# Autodesk Inventor assembly: TankFlipperAssembledDriveShaft
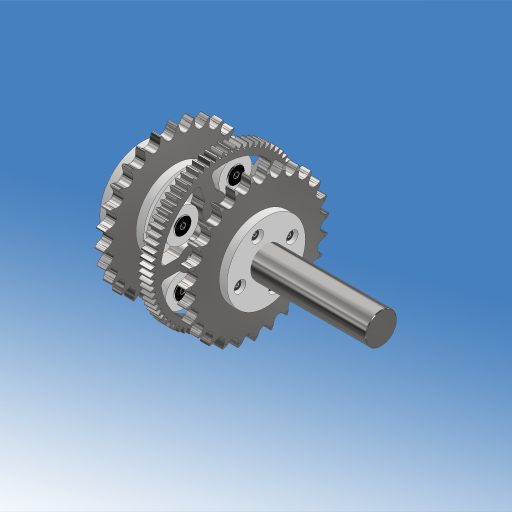
[picture p0: Inventor's stored thumbnail of the model, 512x512]
Saved by Autodesk Inventor 2024 (Build 280153000, 153)
## iProperties
Created: 2024-02-13
Part Number: TankFlipperAssembledDriveShaft
Document SubType Name: Assembly
Designer: seene
Author: seene
## Documents named in this file (12)
- C:\Users\seene\OneDrive\SBRT\Robocup Rescue\Drive\v1\TANK flipper\TankFlipperAssembledDriveShaft.iam
- C:\Users\seene\OneDrive\SBRT\Robocup Rescue\Drive\v1\TANK flipper\Drive Shaft.ipt
- C:\Users\seene\OneDrive\SBRT\Robocup Rescue\Drive\v1\TANK flipper\98585A121_Heavy Duty External Retaining Ring v2.ipt
- C:\Users\seene\OneDrive\SBRT\Robocup Rescue\Drive\v1\TANK flipper\2868T199_High-Load Oil-Embedded 863 Sleeve Bearing (1) v2(Mirror).ipt
- C:\Users\seene\OneDrive\SBRT\Robocup Rescue\Drive\v1\TANK flipper\27t track drive sprocket v25.iam
- C:\Users\seene\OneDrive\SBRT\Robocup Rescue\Drive\v1\TANK flipper\Spur Gear (74 teeth).ipt
- C:\Users\seene\OneDrive\SBRT\Robocup Rescue\Drive\v1\TANK flipper\panel_flange.ipt
- C:\Users\seene\Downloads\SBRT\SBRT\Flipper_assy\spacer_flange.ipt
- C:\Users\seene\OneDrive\SBRT\Robocup Rescue\Drive\v1\TANK flipper\transfer_pin.ipt
- C:\Users\seene\OneDrive\SBRT\Robocup Rescue\Drive\v1\TANK flipper\.25-20_FHCS_91263A553.ipt
- C:\Users\seene\OneDrive\SBRT\Robocup Rescue\Drive\v1\TANK flipper\bushing_2868T199.ipt
- C:\Users\seene\OneDrive\SBRT\Robocup Rescue\Drive\v1\TANK flipper\94328A911_Black Oxide Alloy Steel Low-Profile Shoulder Screw v2.ipt
## Components (29 placed, 11 different names)
1. Drive Shaft:1 — Rigid:1, Rigid:2, Rigid:3, Rigid:4, Rigid:5, Rigid:17
2. 98585A121_Heavy Duty External Retaining Ring v2:1 — Rigid:1
3. 2868T199_High-Load Oil-Embedded 863 Sleeve Bearing (1) v2(Mirror):1 — Rigid:2, Rigid:18
4. 27t track drive sprocket v25:1 [sub-assembly] — Rigid:4
5. 98585A121_Heavy Duty External Retaining Ring v2:2 — Rigid:3
6. 98585A121_Heavy Duty External Retaining Ring v2:3 — Rigid:5
7. Spur Gear (74 teeth):1 — Mate:1, Mate:2, Rigid:16
8. panel_flange:1 — Rigid:18
9. panel_flange:2 — Mate:3, Mate:4, Mate:5, Rigid:25
10. spacer_flange:1 — Rigid:6, Rigid:7, Rigid:8, Rigid:9, Rigid:10, Mate:1, Mate:2, Rigid:20, Rigid:21, Rigid:22, Rigid:23, Rigid:24
11. transfer_pin:1 — Rigid:8, Rigid:14
12. transfer_pin:2 — Rigid:9, Rigid:15
13. transfer_pin:3 — Rigid:7, Rigid:13
14. transfer_pin:4 — Rigid:10, Rigid:11
15. transfer_pin:5 — Rigid:6, Rigid:12
16. .25-20_FHCS_91263A553:1 — Rigid:11
17. .25-20_FHCS_91263A553:2 — Rigid:13
18. .25-20_FHCS_91263A553:3 — Rigid:14
19. .25-20_FHCS_91263A553:4 — Rigid:15
20. .25-20_FHCS_91263A553:5 — Rigid:12
21. bushing_2868T199:1 — Rigid:16, Rigid:26
22. bushing_2868T199:2 — Rigid:26, Rotational:1
23. bushing_2868T199:3 — Rigid:17, Rigid:25
24. 94328A911_Black Oxide Alloy Steel Low-Profile Shoulder Screw v2:1 — Rigid:23, Mate:5
25. 94328A911_Black Oxide Alloy Steel Low-Profile Shoulder Screw v2:2 — Rigid:24
26. 94328A911_Black Oxide Alloy Steel Low-Profile Shoulder Screw v2:3 — Rigid:20
27. 94328A911_Black Oxide Alloy Steel Low-Profile Shoulder Screw v2:4 — Rigid:21, Mate:3, Mate:4
28. 94328A911_Black Oxide Alloy Steel Low-Profile Shoulder Screw v2:5 — Rigid:22
29. 27t track drive sprocket v25:2 [sub-assembly] — Rotational:1
## Relationships (31: WeldJoint 25, Mate 5, RevoluteJoint 1)
- Rigid:1 [WeldJoint]: Drive Shaft:1 ↔ 98585A121_Heavy Duty External Retaining Ring v2:1
- Rigid:2 [WeldJoint]: Drive Shaft:1 ↔ 2868T199_High-Load Oil-Embedded 863 Sleeve Bearing (1) v2(Mirror):1
- Rigid:3 [WeldJoint]: Drive Shaft:1 ↔ 98585A121_Heavy Duty External Retaining Ring v2:2
- Rigid:4 [WeldJoint]: Drive Shaft:1 ↔ 27t track drive sprocket v25:1
- Rigid:5 [WeldJoint]: Drive Shaft:1 ↔ 98585A121_Heavy Duty External Retaining Ring v2:3
- Rigid:6 [WeldJoint]: spacer_flange:1 ↔ transfer_pin:5
- Rigid:7 [WeldJoint]: spacer_flange:1 ↔ transfer_pin:3
- Rigid:8 [WeldJoint]: spacer_flange:1 ↔ transfer_pin:1
- Rigid:9 [WeldJoint]: spacer_flange:1 ↔ transfer_pin:2
- Rigid:10 [WeldJoint]: spacer_flange:1 ↔ transfer_pin:4
- Mate:1: Spur Gear (74 teeth):1 ↔ spacer_flange:1
- Mate:2: Spur Gear (74 teeth):1 ↔ spacer_flange:1
- Rigid:11 [WeldJoint]: transfer_pin:4 ↔ .25-20_FHCS_91263A553:1
- Rigid:12 [WeldJoint]: transfer_pin:5 ↔ .25-20_FHCS_91263A553:5
- Rigid:13 [WeldJoint]: transfer_pin:3 ↔ .25-20_FHCS_91263A553:2
- Rigid:14 [WeldJoint]: transfer_pin:1 ↔ .25-20_FHCS_91263A553:3
- Rigid:15 [WeldJoint]: transfer_pin:2 ↔ .25-20_FHCS_91263A553:4
- Rigid:16 [WeldJoint]: Spur Gear (74 teeth):1 ↔ bushing_2868T199:1
- Rigid:17 [WeldJoint]: Drive Shaft:1 ↔ bushing_2868T199:3
- Rigid:18 [WeldJoint]: 2868T199_High-Load Oil-Embedded 863 Sleeve Bearing (1) v2(Mirror):1 ↔ panel_flange:1
- Rigid:20 [WeldJoint]: spacer_flange:1 ↔ 94328A911_Black Oxide Alloy Steel Low-Profile Shoulder Screw v2:3
- Rigid:21 [WeldJoint]: spacer_flange:1 ↔ 94328A911_Black Oxide Alloy Steel Low-Profile Shoulder Screw v2:4
- Rigid:22 [WeldJoint]: spacer_flange:1 ↔ 94328A911_Black Oxide Alloy Steel Low-Profile Shoulder Screw v2:5
- Rigid:23 [WeldJoint]: spacer_flange:1 ↔ 94328A911_Black Oxide Alloy Steel Low-Profile Shoulder Screw v2:1
- Rigid:24 [WeldJoint]: spacer_flange:1 ↔ 94328A911_Black Oxide Alloy Steel Low-Profile Shoulder Screw v2:2
- Mate:3: panel_flange:2 ↔ 94328A911_Black Oxide Alloy Steel Low-Profile Shoulder Screw v2:4
- Mate:4: panel_flange:2 ↔ 94328A911_Black Oxide Alloy Steel Low-Profile Shoulder Screw v2:4
- Mate:5: panel_flange:2 ↔ 94328A911_Black Oxide Alloy Steel Low-Profile Shoulder Screw v2:1
- Rigid:25 [WeldJoint]: panel_flange:2 ↔ bushing_2868T199:3
- Rigid:26 [WeldJoint]: bushing_2868T199:1 ↔ bushing_2868T199:2
- Rotational:1 [RevoluteJoint]: bushing_2868T199:2 ↔ 27t track drive sprocket v25:2
